# Autodesk Inventor assembly: Rrwing cost
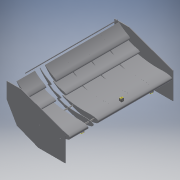
[picture p0: Inventor's stored thumbnail of the model, 180x180]
Saved by Autodesk Inventor 2018.3 (Build 223284000, 284)
## iProperties
Created: 2018-06-13
Part Number: Rrwing cost
Material: 一般
Document SubType Name: Assembly
Designer: ku_sk
Author: ku_sk
## Documents named in this file (12)
- D:\ku_sk\ドキュメント\Inventor\Aero\KS-15\コスト用CAD\Rrwing\Rrwing cost.iam
- D:\ku_sk\ドキュメント\Inventor\Aero\KS-15\コスト用CAD\Rrwing\parts\endplate.ipt
- D:\ku_sk\ドキュメント\Inventor\Aero\KS-15\コスト用CAD\Rrwing\parts\mainflap.ipt
- D:\ku_sk\ドキュメント\Inventor\Aero\KS-15\コスト用CAD\Rrwing\parts\splitter.ipt
- D:\ku_sk\ドキュメント\Inventor\Aero\KS-15\コスト用CAD\Rrwing\parts\subflap.ipt
- D:\ku_sk\ドキュメント\Inventor\Aero\KS-15\コスト用CAD\Rrwing\parts\mainflap for center.ipt
- D:\ku_sk\ドキュメント\Inventor\Aero\KS-15\コスト用CAD\Rrwing\parts\mainflap for side L.ipt
- D:\ku_sk\ドキュメント\Inventor\Aero\KS-15\コスト用CAD\Rrwing\parts\mainflap for side R.ipt
- D:\ku_sk\ドキュメント\Inventor\Aero\KS-15\コスト用CAD\Rrwing\parts\core.ipt
- D:\ku_sk\ドキュメント\Inventor\Aero\KS-15\コスト用CAD\Rrwing\parts\bracket FU RL.ipt
- D:\ku_sk\ドキュメント\Inventor\Aero\KS-15\コスト用CAD\Rrwing\parts\bracket FL.ipt
- D:\ku_sk\ドキュメント\Inventor\Aero\KS-15\コスト用CAD\Rrwing\parts\gurnee.ipt
## Components (29 placed, 11 different names)
1. endplate:1 — メイト:1, メイト:2, メイト:3, 角度:1
2. mainflap:1 — フラッシュ:1, メイト:2, メイト:3, メイト:4, メイト:5, メイト:6, メイト:10, メイト:11, メイト:12, フラッシュ:3
3. splitter:1 — メイト:10, メイト:11, メイト:12, メイト:21, メイト:22, メイト:46, メイト:47, メイト:54, メイト:55
4. subflap:1 — メイト:21, メイト:22, フラッシュ:3, フラッシュ:8
5. endplate:2 — メイト:58, メイト:59, メイト:60, メイト:80
6. splitter:2 — メイト:23, メイト:24, メイト:28, メイト:29, メイト:34, メイト:40, メイト:41, メイト:48, メイト:49, メイト:56
7. subflap:2 — メイト:19, メイト:20, フラッシュ:7
8. splitter:3 — メイト:4, メイト:5, メイト:6, メイト:19, メイト:20, メイト:44, メイト:45, メイト:57, メイト:61, メイト:62
9. subflap:3 — メイト:23, メイト:24, フラッシュ:9
10. mainflap:4 — メイト:28, メイト:29, メイト:32, メイト:33, メイト:34, メイト:35, フラッシュ:5
11. subflap:4 — メイト:40, メイト:41, フラッシュ:5, フラッシュ:10
12. subflap:5 — メイト:42, メイト:43
13. splitter:4 — メイト:32, メイト:33, メイト:35, メイト:42, メイト:43, メイト:50, メイト:51, メイト:52, メイト:53
14. subflap:6 — メイト:44, メイト:45, フラッシュ:7
15. subflap:7 — メイト:46, メイト:47, フラッシュ:8
16. subflap:8 — メイト:48, メイト:49, フラッシュ:9
17. subflap:9 — メイト:50, メイト:51, フラッシュ:10, 正接:1
18. subflap:10 — メイト:52, メイト:53
19. mainflap for center:1 — メイト:54, メイト:55, メイト:56, メイト:66, メイト:67
20. mainflap for side L:1 — メイト:58, メイト:59, メイト:60, メイト:69, メイト:70, メイト:75, メイト:76
21. mainflap for side R:1 — メイト:57, メイト:61, メイト:62, メイト:63, メイト:64, フラッシュ:12, メイト:72, メイト:73, メイト:78, メイト:79
22. core:1 — メイト:63, フラッシュ:11, メイト:68, メイト:71
23. core:2 — メイト:64, フラッシュ:11, フラッシュ:12, メイト:65, メイト:74, メイト:77
24. bracket FU RL:1 — メイト:65, メイト:66, メイト:67
25. bracket FU RL:2 — メイト:71, メイト:72, メイト:73
26. bracket FU RL:3 — メイト:68, メイト:69, メイト:70
27. bracket FL:1 — メイト:74, メイト:75, メイト:76
28. bracket FL:2 — メイト:77, メイト:78, メイト:79
29. gurnee:1 — 正接:1, メイト:80
## Relationships (73: Mate 62, Flush 9, Angle 1, Tangent 1)
- メイト:1 [Mate]: endplate:1
- フラッシュ:1 [Flush]: mainflap:1
- メイト:2 [Mate]: endplate:1 ↔ mainflap:1
- メイト:3 [Mate]: endplate:1 ↔ mainflap:1
- 角度:1 [Angle] (0 deg): endplate:1
- メイト:4 [Mate]: mainflap:1 ↔ splitter:3
- メイト:5 [Mate]: mainflap:1 ↔ splitter:3
- メイト:6 [Mate] (50 mm): mainflap:1 ↔ splitter:3
- メイト:10 [Mate]: mainflap:1 ↔ splitter:1
- メイト:11 [Mate]: mainflap:1 ↔ splitter:1
- メイト:12 [Mate]: mainflap:1 ↔ splitter:1
- メイト:19 [Mate]: subflap:2 ↔ splitter:3
- メイト:20 [Mate]: subflap:2 ↔ splitter:3
- メイト:21 [Mate]: splitter:1 ↔ subflap:1
- メイト:22 [Mate]: splitter:1 ↔ subflap:1
- メイト:23 [Mate]: splitter:2 ↔ subflap:3
- メイト:24 [Mate]: splitter:2 ↔ subflap:3
- フラッシュ:3 [Flush]: mainflap:1 ↔ subflap:1
- メイト:28 [Mate]: splitter:2 ↔ mainflap:4
- メイト:29 [Mate]: splitter:2 ↔ mainflap:4
- メイト:32 [Mate]: mainflap:4 ↔ splitter:4
- メイト:33 [Mate]: mainflap:4 ↔ splitter:4
- メイト:34 [Mate]: splitter:2 ↔ mainflap:4
- メイト:35 [Mate]: mainflap:4 ↔ splitter:4
- メイト:40 [Mate]: splitter:2 ↔ subflap:4
- メイト:41 [Mate]: splitter:2 ↔ subflap:4
- メイト:42 [Mate]: subflap:5 ↔ splitter:4
- メイト:43 [Mate]: subflap:5 ↔ splitter:4
- フラッシュ:5 [Flush]: mainflap:4 ↔ subflap:4
- メイト:44 [Mate]: splitter:3 ↔ subflap:6
- メイト:45 [Mate]: splitter:3 ↔ subflap:6
- フラッシュ:7 [Flush]: subflap:2 ↔ subflap:6
- メイト:46 [Mate]: splitter:1 ↔ subflap:7
- メイト:47 [Mate]: splitter:1 ↔ subflap:7
- フラッシュ:8 [Flush]: subflap:1 ↔ subflap:7
- メイト:48 [Mate]: splitter:2 ↔ subflap:8
- メイト:49 [Mate]: splitter:2 ↔ subflap:8
- メイト:50 [Mate]: splitter:4 ↔ subflap:9
- メイト:51 [Mate]: splitter:4 ↔ subflap:9
- フラッシュ:9 [Flush]: subflap:3 ↔ subflap:8
- フラッシュ:10 [Flush]: subflap:4 ↔ subflap:9
- メイト:52 [Mate]: splitter:4 ↔ subflap:10
- メイト:53 [Mate]: splitter:4 ↔ subflap:10
- メイト:54 [Mate]: splitter:1 ↔ mainflap for center:1
- メイト:55 [Mate]: splitter:1 ↔ mainflap for center:1
- メイト:56 [Mate]: splitter:2 ↔ mainflap for center:1
- メイト:57 [Mate]: splitter:3 ↔ mainflap for side R:1
- メイト:58 [Mate]: endplate:2 ↔ mainflap for side L:1
- メイト:59 [Mate]: endplate:2 ↔ mainflap for side L:1
- メイト:60 [Mate]: endplate:2 ↔ mainflap for side L:1
- メイト:61 [Mate]: splitter:3 ↔ mainflap for side R:1
- メイト:62 [Mate] (50 mm): splitter:3 ↔ mainflap for side R:1
- メイト:63 [Mate]: mainflap for side R:1 ↔ core:1
- メイト:64 [Mate]: mainflap for side R:1 ↔ core:2
- フラッシュ:11 [Flush]: core:1 ↔ core:2
- フラッシュ:12 [Flush] (-25 mm): mainflap for side R:1 ↔ core:2
- メイト:65 [Mate]: core:2 ↔ bracket FU RL:1
- メイト:66 [Mate] (1 mm): mainflap for center:1 ↔ bracket FU RL:1
- メイト:67 [Mate] (1 mm): mainflap for center:1 ↔ bracket FU RL:1
- メイト:68 [Mate]: core:1 ↔ bracket FU RL:3
- メイト:69 [Mate] (1 mm): mainflap for side L:1 ↔ bracket FU RL:3
- メイト:70 [Mate] (1 mm): mainflap for side L:1 ↔ bracket FU RL:3
- メイト:71 [Mate]: core:1 ↔ bracket FU RL:2
- メイト:72 [Mate] (1 mm): mainflap for side R:1 ↔ bracket FU RL:2
- メイト:73 [Mate] (1 mm): mainflap for side R:1 ↔ bracket FU RL:2
- メイト:74 [Mate]: core:2 ↔ bracket FL:1
- メイト:75 [Mate] (1 mm): mainflap for side L:1 ↔ bracket FL:1
- メイト:76 [Mate] (1 mm): mainflap for side L:1 ↔ bracket FL:1
- メイト:77 [Mate]: core:2 ↔ bracket FL:2
- メイト:78 [Mate] (1 mm): mainflap for side R:1 ↔ bracket FL:2
- メイト:79 [Mate] (1 mm): mainflap for side R:1 ↔ bracket FL:2
- 正接:1 [Tangent]: subflap:9 ↔ gurnee:1
- メイト:80 [Mate]: endplate:2 ↔ gurnee:1
